# Autodesk Inventor assembly: 200 rpm motor assembly
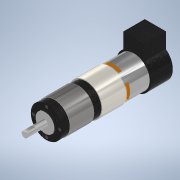
[picture p0: Inventor's stored thumbnail of the model, 180x180]
Saved by Autodesk Inventor 2020 (Build 240168000, 168)
## iProperties
Created: 2020-07-27
Part Number: 200 rpm motor assembly
Document SubType Name: Assembly
Designer: Ashiqrahman
Author: Ashiqrahman
## Documents named in this file (3)
- D:\projects\Intelligent Picking\my models\200 rpm motor assembly.iam
- C:\Users\Public\Documents\Autodesk\Inventor 2020\motorbody.ipt
- C:\Users\Public\Documents\Autodesk\Inventor 2020\motor_shaft.ipt
## Components (2 placed, 2 different names)
1. motorbody:1 — Flush:1, Mate:1
2. motor_shaft:1 — Flush:1, Mate:1
## Relationships (2: Flush 1, Mate 1)
- Flush:1: motorbody:1 ↔ motor_shaft:1
- Mate:1: motorbody:1 ↔ motor_shaft:1
